# Autodesk Inventor assembly: Assembly1
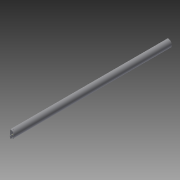
[picture p0: Inventor's stored thumbnail of the model, 180x180]
Saved by Autodesk Inventor 2015 SP1 (Build 190203100, 203)
## iProperties
Created: 2015-03-28
Part Number: Assembly1
Document SubType Name: Assembly
Designer: Cyril
Mass: 815.005 g
Surface Area: 4323.83 cm^2
Volume: 815.005 cm^3
Density: 1 g/cm^3
Author: Cyril
## Documents named in this file (11)
- C:\Users\Cyril\Documents\OSE FR\Concentrateur solaire\Assemblage_mirroir.iam
- C:\Users\Cyril\Documents\OSE FR\Concentrateur solaire\Mirroir.ipt
- C:\Users\Cyril\Documents\OSE FR\Concentrateur solaire\Part3.ipt
- C:\Users\Cyril\Documents\OSE FR\Concentrateur solaire\Tube sous miroir.ipt
- C:\Users\Cyril\Documents\OSE FR\Concentrateur solaire\tige.ipt
- C:\Users\Cyril\Documents\OSE FR\Concentrateur solaire\ecrou_nf_en_iso_4032_m4_6.ipt
- C:\Users\Cyril\Documents\OSE FR\Concentrateur solaire\Mirroir_MIR.ipt
- C:\Users\Cyril\Documents\OSE FR\Concentrateur solaire\Part3_MIR.ipt
- C:\Users\Cyril\Documents\OSE FR\Concentrateur solaire\Tube sous miroir_MIR.ipt
- C:\Users\Cyril\Documents\OSE FR\Concentrateur solaire\tige_MIR.ipt
- C:\Users\Cyril\Documents\OSE FR\Concentrateur solaire\ecrou_nf_en_iso_4032_m4_6_MIR.ipt
## Components (10 placed, 10 different names)
1. Mirroir:1 — Flush:4, Mate:13, Mate:14, Angle:1
2. Part3:1 — Mate:17, Flush:5, Flush:6, Angle:1
3. Tube sous miroir:1 — Flush:4, Mate:13, Mate:14, Mate:15, Mate:16, Flush:5
4. tige:1 — Mate:15, Mate:16, Mate:17, Mate:18
5. ecrou_nf_en_iso_4032_m4_6:1 — Mate:18, Flush:6
6. Mirroir_MIR:1 — Angle:2, Mate:19, Mate:20, Flush:8
7. Part3_MIR:1 — Angle:2, Flush:7, Mate:21, Flush:10
8. Tube sous miroir_MIR:1 — Flush:7, Mate:19, Mate:20, Flush:8, Flush:9, Mate:22
9. tige_MIR:1 — Mate:21, Flush:9, Mate:22, Mate:23
10. ecrou_nf_en_iso_4032_m4_6_MIR:1 — Flush:10, Mate:23
## Relationships (20: Mate 11, Flush 7, Angle 2)
- Flush:4: Mirroir:1 ↔ Tube sous miroir:1
- Mate:13: Mirroir:1 ↔ Tube sous miroir:1
- Mate:14: Mirroir:1 ↔ Tube sous miroir:1
- Mate:15: Tube sous miroir:1 ↔ tige:1
- Mate:16: Tube sous miroir:1 ↔ tige:1
- Mate:17: Part3:1 ↔ tige:1
- Flush:5: Part3:1 ↔ Tube sous miroir:1
- Mate:18: tige:1 ↔ ecrou_nf_en_iso_4032_m4_6:1
- Flush:6 (47.2 mm): Part3:1 ↔ ecrou_nf_en_iso_4032_m4_6:1
- Angle:1 (0 deg): Mirroir:1 ↔ Part3:1
- Angle:2 (0 deg): Mirroir_MIR:1 ↔ Part3_MIR:1
- Flush:7: Part3_MIR:1 ↔ Tube sous miroir_MIR:1
- Mate:19: Mirroir_MIR:1 ↔ Tube sous miroir_MIR:1
- Mate:20: Mirroir_MIR:1 ↔ Tube sous miroir_MIR:1
- Flush:8: Mirroir_MIR:1 ↔ Tube sous miroir_MIR:1
- Mate:21: Part3_MIR:1 ↔ tige_MIR:1
- Flush:9: Tube sous miroir_MIR:1 ↔ tige_MIR:1
- Mate:22: Tube sous miroir_MIR:1 ↔ tige_MIR:1
- Flush:10 (47.2 mm): Part3_MIR:1 ↔ ecrou_nf_en_iso_4032_m4_6_MIR:1
- Mate:23: tige_MIR:1 ↔ ecrou_nf_en_iso_4032_m4_6_MIR:1
